# Autodesk Inventor assembly: Camera+Adapter+Filterwheel+Poles
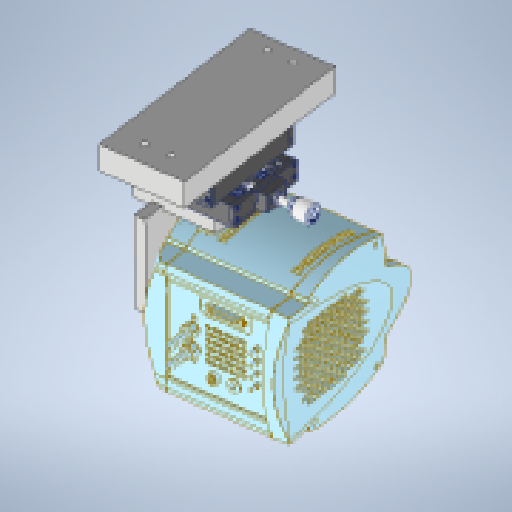
[picture p0: Inventor's stored thumbnail of the model, 512x512]
Saved by Autodesk Inventor 2026.1 (Build 301233000, 233)
## iProperties
Created: 2019-05-03
Part Number: Camera+Adapter+Filterwheel+Poles
Document SubType Name: Assembly
Designer: Administrator
Author: Administrator
## Documents named in this file (7)
- C:\Users\user\Desktop\setup for publishing\Camera+Adapter+Filterwheel+Poles.iam
- C:\Users\user\Desktop\setup for publishing\Andor_Carmera+MountInfo.ipt
- C:\Users\user\Desktop\setup for publishing\SM1toC-Mount.ipt
- C:\Users\user\Desktop\setup for publishing\PT1B_M_TranslationalStage.ipt
- C:\Users\user\Desktop\setup for publishing\CameraAdapter_part1.ipt
- C:\Users\user\Desktop\setup for publishing\CameraAdapter_part2.ipt
- C:\Users\user\Desktop\setup for publishing\CameraAdapter_part3.ipt
## Components (7 placed, 6 different names)
1. Andor_Carmera+MountInfo:1 — Passend:13, Passend:14, Passend:21, Passend:22, Passend:38
2. SM1toC-Mount:1 — Passend:13, Passend:14
3. PT1B_M_TranslationalStage:1 — Passend:15, Passend:16, Winkel:1, Passend:25, Passend:26, Passend:27
4. PT1B_M_TranslationalStage:2 — Passend:15, Passend:16, Winkel:1, Passend:23, Passend:24, Winkel:4
5. CameraAdapter_part1:1 — Passend:18, Passend:21, Passend:22, Passend:23, Passend:24, Winkel:4, Passend:28, Passend:29
6. CameraAdapter_part2:1 — Passend:18, Passend:28, Passend:29, Winkel:5
7. CameraAdapter_part3:1 — Passend:25, Passend:26, Passend:27
## Relationships (18: Mate 15, Angle 3)
- Passend:13 [Mate]: Andor_Carmera+MountInfo:1 ↔ SM1toC-Mount:1
- Passend:14 [Mate]: Andor_Carmera+MountInfo:1 ↔ SM1toC-Mount:1
- Passend:15 [Mate]: PT1B_M_TranslationalStage:1 ↔ PT1B_M_TranslationalStage:2
- Passend:16 [Mate]: PT1B_M_TranslationalStage:1 ↔ PT1B_M_TranslationalStage:2
- Winkel:1 [Angle] (0 deg): PT1B_M_TranslationalStage:1 ↔ PT1B_M_TranslationalStage:2
- Passend:18 [Mate]: CameraAdapter_part1:1 ↔ CameraAdapter_part2:1
- Passend:21 [Mate] (-9.8 mm): Andor_Carmera+MountInfo:1 ↔ CameraAdapter_part1:1
- Passend:22 [Mate]: Andor_Carmera+MountInfo:1 ↔ CameraAdapter_part1:1
- Passend:23 [Mate]: PT1B_M_TranslationalStage:2 ↔ CameraAdapter_part1:1
- Passend:24 [Mate]: PT1B_M_TranslationalStage:2 ↔ CameraAdapter_part1:1
- Winkel:4 [Angle] (0 deg): PT1B_M_TranslationalStage:2 ↔ CameraAdapter_part1:1
- Passend:25 [Mate]: PT1B_M_TranslationalStage:1 ↔ CameraAdapter_part3:1
- Passend:26 [Mate]: PT1B_M_TranslationalStage:1 ↔ CameraAdapter_part3:1
- Passend:27 [Mate]: PT1B_M_TranslationalStage:1 ↔ CameraAdapter_part3:1
- Passend:28 [Mate]: CameraAdapter_part1:1 ↔ CameraAdapter_part2:1
- Passend:29 [Mate]: CameraAdapter_part1:1 ↔ CameraAdapter_part2:1
- Passend:38 [Mate]: Andor_Carmera+MountInfo:1
- Winkel:5 [Angle] (90 deg): CameraAdapter_part2:1
